# Autodesk Inventor assembly: trencompleto
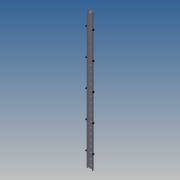
[picture p0: Inventor's stored thumbnail of the model, 180x180]
Saved by Autodesk Inventor 2011 (Build 150239000, 239)
## iProperties
Created: 2011-09-24
Part Number: trencompleto
Document SubType Name: Assembly
Designer: mgaspari
Author: mgaspari
## Documents named in this file (3)
- C:\Users\IBM_ADMIN\Desktop\cilindro\Mio\Guia\trencompleto.iam
- C:\Users\IBM_ADMIN\Desktop\cilindro\Mio\Guia\tren.ipt
- C:\Users\IBM_ADMIN\Desktop\cilindro\Mio\Guia\falsarueda.ipt
## Components (11 placed, 2 different names)
1. tren:1 — Insert:1, Insert:2, Insert:3, Insert:4, Insert:5, Insert:6, Insert:7, Insert:8, Insert:9, Insert:10
2. falsarueda:1 — Insert:1
3. falsarueda:2 — Insert:2
4. falsarueda:3 — Insert:5
5. falsarueda:4 — Insert:3
6. falsarueda:5 — Insert:9
7. falsarueda:6 — Insert:7
8. falsarueda:7 — Insert:4
9. falsarueda:8 — Insert:6
10. falsarueda:9 — Insert:10
11. falsarueda:10 — Insert:8
## Relationships (10: Insert 10)
- Insert:1 (-1 mm): tren:1 ↔ falsarueda:1
- Insert:2 (-1 mm): tren:1 ↔ falsarueda:2
- Insert:3 (-1 mm): tren:1 ↔ falsarueda:4
- Insert:4 (-1 mm): tren:1 ↔ falsarueda:7
- Insert:5 (-1 mm): tren:1 ↔ falsarueda:3
- Insert:6 (-1 mm): tren:1 ↔ falsarueda:8
- Insert:7 (-1 mm): tren:1 ↔ falsarueda:6
- Insert:8 (-1 mm): tren:1 ↔ falsarueda:10
- Insert:9 (-1 mm): tren:1 ↔ falsarueda:5
- Insert:10 (-1 mm): tren:1 ↔ falsarueda:9
